# Autodesk Inventor assembly: Shim_cartridge_V4_template
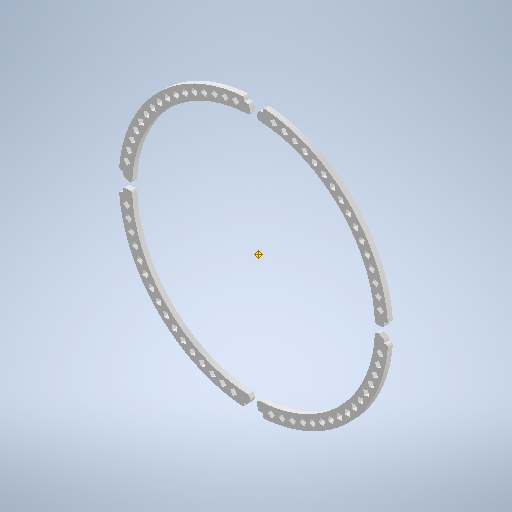
[picture p0: Inventor's stored thumbnail of the model, 512x512]
Saved by Autodesk Inventor 2025.2 (Build 292293000, 293)
## iProperties
Created: 2025-04-15
Part Number: Shim_cartridge_V4_template
Document SubType Name: Assembly
Designer: Joshua Harper
Author: Joshua Harper
## Documents named in this file (2)
- C:\Users\Carla Fernandez\Documents\GitHub\OSII_MINI_V2\CAD MODELS\Shim_cartridge_V4_template.iam
- C:\Users\Carla Fernandez\Documents\GitHub\OSII_MINI_V2\CAD MODELS\shim_cartridge_V4.ipt
## Components (4 placed, 1 different names)
1. shim_cartridge_V4:1 — Flush:1, Flush:4, Flush:5, Mate:3
2. shim_cartridge_V4:2 — Flush:2, Flush:3, Flush:5, Mate:3, Mate:4
3. shim_cartridge_V4:3 — Flush:3, Mate:1, Mate:4, Mate:5, Mate:6
4. shim_cartridge_V4:4 — Mate:2, Flush:4, Mate:5
## Relationships (11: Mate 6, Flush 5)
- Flush:1: shim_cartridge_V4:1
- Flush:2: shim_cartridge_V4:2
- Flush:3: shim_cartridge_V4:2 ↔ shim_cartridge_V4:3
- Mate:1: shim_cartridge_V4:3
- Mate:2: shim_cartridge_V4:4
- Flush:4: shim_cartridge_V4:1 ↔ shim_cartridge_V4:4
- Flush:5: shim_cartridge_V4:1 ↔ shim_cartridge_V4:2
- Mate:3: shim_cartridge_V4:1 ↔ shim_cartridge_V4:2
- Mate:4: shim_cartridge_V4:2 ↔ shim_cartridge_V4:3
- Mate:5: shim_cartridge_V4:3 ↔ shim_cartridge_V4:4
- Mate:6: shim_cartridge_V4:3
